# Autodesk Inventor assembly: stojak
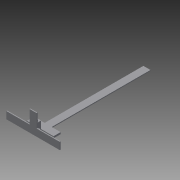
[picture p0: Inventor's stored thumbnail of the model, 180x180]
Saved by Autodesk Inventor 2014 (Build 180170000, 170)
## iProperties
Created: 2014-12-22
Part Number: stojak
Document SubType Name: Assembly
Designer: Kuba
Author: Kuba
## Documents named in this file (10)
- C:\Users\Kuba\Dysk Google\synergia\RoboDrift2015\Pomiar czasu\konstrukcja\stojak.iam
- C:\Users\Kuba\Dysk Google\synergia\RoboDrift2015\Pomiar czasu\konstrukcja\podstawa d.ipt
- C:\Users\Kuba\Dysk Google\synergia\RoboDrift2015\Pomiar czasu\konstrukcja\czujnik.ipt
- C:\Users\Kuba\Dysk Google\synergia\RoboDrift2015\Pomiar czasu\konstrukcja\podstawa krótka.ipt
- C:\Users\Kuba\Dysk Google\synergia\RoboDrift2015\Pomiar czasu\konstrukcja\płaskownik.ipt
- C:\Users\Kuba\Documents\Inventor\Content Center Files\R2014\pl-PL\ISO 7050 - C-Z(1)\ISO 7050 - ST4,8 x 9,5 - C - ZDIN ISO.ipt
- C:\Users\Kuba\Dysk Google\synergia\RoboDrift2015\Pomiar czasu\konstrukcja\DIN EN 10056-1 - L60x60x5-40.ipt
- C:\Users\Kuba\Dysk Google\synergia\RoboDrift2015\Pomiar czasu\konstrukcja\deska300x80.ipt
- C:\Users\Kuba\Dysk Google\synergia\RoboDrift2015\Pomiar czasu\konstrukcja\deska120x80.ipt
- C:\Users\Kuba\Dysk Google\synergia\RoboDrift2015\Pomiar czasu\konstrukcja\listwa20x20x50.ipt
## Components (19 placed, 10 different names)
1. podstawa d:1 — Zestawiający:1, Zestawiający:2, Równoległy:1, Równoległy:2, Zestawiający:3, Zestawiający:4, Zestawiający:5, Zestawiający:6, Równoległy:5, Zestawiający:8, Równoległy:9, Zestawiający:10, Zestawiający:15, Równoległy:15, Równoległy:16, Zestawiający:16
2. czujnik:1 — Równoległy:2, Zestawiający:3, Równoległy:4, Zestawiający:17, Zestawiający:18, Zestawiający:20
3. deska 150x80 — Zestawiający:1, Zestawiający:2, Równoległy:1, Równoległy:3, Równoległy:4, Zestawiający:12, Zestawiający:14, Zestawiający:19, Równoległy:17
4. płaskownik:1 — Zestawiający:4, Zestawiający:5, Równoległy:3, Wstaw:1, Wstaw:2, Wstaw:3, Wstaw:4, Wstaw:5, Wstaw:6
5. DIN ISO 7050 - C-Z ST4,8 x 9,5 - C - Z:1 — Wstaw:1
6. DIN ISO 7050 - C-Z ST4,8 x 9,5 - C - Z:2 — Wstaw:2
7. DIN ISO 7050 - C-Z ST4,8 x 9,5 - C - Z:3 — Wstaw:3
8. DIN ISO 7050 - C-Z ST4,8 x 9,5 - C - Z:4 — Wstaw:4
9. DIN ISO 7050 - C-Z ST4,8 x 9,5 - C - Z:5 — Wstaw:6
10. DIN ISO 7050 - C-Z ST4,8 x 9,5 - C - Z:6 — Wstaw:5
11. DIN EN 10056-1 - L60x60x5-40:1 — Zestawiający:6, Równoległy:5, Zestawiający:7, Równoległy:6
12. podstawa krótka:2 — Zestawiający:7, Zestawiający:8, Równoległy:6, Zestawiający:11, Równoległy:11, Równoległy:12
13. DIN EN 10056-1 - L60x60x5-40:2 — Równoległy:8, Zestawiający:10
14. podstawa krótka:3 — Równoległy:8, Równoległy:9, Równoległy:10
15. deska300x80:1 — Zestawiający:11, Równoległy:10, Równoległy:11, Równoległy:12, Zestawiający:12, Równoległy:14, Zestawiający:13
16. deska120x80:1 — Równoległy:14, Zestawiający:13, Zestawiający:14
17. listwa20x20x50:1 — Zestawiający:15, Równoległy:15, Zestawiający:18
18. listwa20x20x50:2 — Równoległy:16, Zestawiający:16, Zestawiający:17
19. listwa20x20x50:3 — Zestawiający:19, Zestawiający:20, Równoległy:17
## Relationships (42: Mate 20, Flush 16, Insert 6)
- Zestawiający:1 [Mate]: podstawa d:1 ↔ deska 150x80
- Zestawiający:2 [Mate]: podstawa d:1 ↔ deska 150x80
- Równoległy:1 [Flush]: podstawa d:1 ↔ deska 150x80
- Równoległy:2 [Flush]: podstawa d:1 ↔ czujnik:1
- Zestawiający:3 [Mate]: podstawa d:1 ↔ czujnik:1
- Zestawiający:4 [Mate]: podstawa d:1 ↔ płaskownik:1
- Zestawiający:5 [Mate]: podstawa d:1 ↔ płaskownik:1
- Równoległy:3 [Flush]: deska 150x80 ↔ płaskownik:1
- Wstaw:1 [Insert] (-4.65 mm): płaskownik:1 ↔ DIN ISO 7050 - C-Z ST4,8 x 9,5 - C - Z:1
- Wstaw:2 [Insert] (-2.25 mm): płaskownik:1 ↔ DIN ISO 7050 - C-Z ST4,8 x 9,5 - C - Z:2
- Wstaw:3 [Insert] (-2.25 mm): płaskownik:1 ↔ DIN ISO 7050 - C-Z ST4,8 x 9,5 - C - Z:3
- Wstaw:4 [Insert] (-4.65 mm): płaskownik:1 ↔ DIN ISO 7050 - C-Z ST4,8 x 9,5 - C - Z:4
- Wstaw:5 [Insert] (-2.25 mm): płaskownik:1 ↔ DIN ISO 7050 - C-Z ST4,8 x 9,5 - C - Z:6
- Wstaw:6 [Insert] (-4.65 mm): płaskownik:1 ↔ DIN ISO 7050 - C-Z ST4,8 x 9,5 - C - Z:5
- Równoległy:4 [Flush]: czujnik:1 ↔ deska 150x80
- Zestawiający:6 [Mate]: podstawa d:1 ↔ DIN EN 10056-1 - L60x60x5-40:1
- Równoległy:5 [Flush] (10 mm): podstawa d:1 ↔ DIN EN 10056-1 - L60x60x5-40:1
- Zestawiający:7 [Mate]: DIN EN 10056-1 - L60x60x5-40:1 ↔ podstawa krótka:2
- Zestawiający:8 [Mate]: podstawa d:1 ↔ podstawa krótka:2
- Równoległy:6 [Flush] (20 mm): DIN EN 10056-1 - L60x60x5-40:1 ↔ podstawa krótka:2
- [Mate]: DIN EN 10056-1 - L60x60x5-40:2 ↔ podstawa krótka:3
- [Flush] (20 mm): DIN EN 10056-1 - L60x60x5-40:2 ↔ podstawa krótka:3
- Równoległy:8 [Flush]: DIN EN 10056-1 - L60x60x5-40:2 ↔ podstawa krótka:3
- Równoległy:9 [Flush]: podstawa d:1 ↔ podstawa krótka:3
- Zestawiający:10 [Mate]: podstawa d:1 ↔ DIN EN 10056-1 - L60x60x5-40:2
- Zestawiający:11 [Mate]: podstawa krótka:2 ↔ deska300x80:1
- Równoległy:10 [Flush]: podstawa krótka:3 ↔ deska300x80:1
- Równoległy:11 [Flush]: podstawa krótka:2 ↔ deska300x80:1
- Równoległy:12 [Flush]: podstawa krótka:2 ↔ deska300x80:1
- Zestawiający:12 [Mate]: deska 150x80 ↔ deska300x80:1
- Równoległy:14 [Flush]: deska300x80:1 ↔ deska120x80:1
- Zestawiający:13 [Mate]: deska300x80:1 ↔ deska120x80:1
- Zestawiający:14 [Mate]: deska 150x80 ↔ deska120x80:1
- Zestawiający:15 [Mate]: podstawa d:1 ↔ listwa20x20x50:1
- Równoległy:15 [Flush] (15 mm): podstawa d:1 ↔ listwa20x20x50:1
- Równoległy:16 [Flush] (15 mm): podstawa d:1 ↔ listwa20x20x50:2
- Zestawiający:16 [Mate]: podstawa d:1 ↔ listwa20x20x50:2
- Zestawiający:17 [Mate]: czujnik:1 ↔ listwa20x20x50:2
- Zestawiający:18 [Mate]: czujnik:1 ↔ listwa20x20x50:1
- Zestawiający:19 [Mate]: deska 150x80 ↔ listwa20x20x50:3
- Zestawiający:20 [Mate]: czujnik:1 ↔ listwa20x20x50:3
- Równoległy:17 [Flush]: deska 150x80 ↔ listwa20x20x50:3
## Named parameters: d25_d22 = 0 mm, d26_d24 = 20 mm
